# Autodesk Inventor assembly: Hotplate Assembly V01
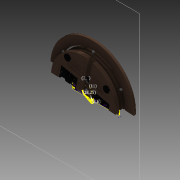
[picture p0: Inventor's stored thumbnail of the model, 180x180]
Saved by Autodesk Inventor 2015 (Build 190159000, 159)
## iProperties
Created: 2016-08-07
Part Number: Hotplate Assembly V01
Document SubType Name: Assembly
Designer: spichelh
Author: spichelh
## Documents named in this file (13)
- C:\Users\spichelh\Documents\GitHub\beta-hardware\Manufacturing Tools\PCB Reflow Hotplate V01\Hotplate Assembly V01.iam
- C:\Users\spichelh\Documents\GitHub\beta-hardware\Manufacturing Tools\PCB Reflow Hotplate V01\Ceramic Heating Element.ipt
- C:\Users\spichelh\Documents\GitHub\beta-hardware\Manufacturing Tools\PCB Reflow Hotplate V01\Hotplate Top 01.ipt
- C:\Users\spichelh\Documents\GitHub\beta-hardware\Manufacturing Tools\PCB Reflow Hotplate V01\HandleTop01.ipt
- C:\Users\spichelh\Documents\GitHub\beta-hardware\Manufacturing Tools\PCB Reflow Bracket V01\PCBBracket01.iam
- C:\Users\spichelh\Documents\GitHub\beta-hardware\Manufacturing Tools\PCB Reflow Hotplate V01\Hotplate Bottom 01.ipt
- C:\Users\spichelh\Documents\GitHub\beta-hardware\Manufacturing Tools\PCB Reflow Hotplate V01\Slippad.ipt
- C:\Users\spichelh\Documents\GitHub\beta-hardware\Manufacturing Tools\PCB Reflow Hotplate V01\HeatingElementHolder01.ipt
- C:\Users\spichelh\Documents\Inventor\Content Center Files\R2015\en-US\JIS B 1111(1)\JIS B 1111 - M2,5x5(1).ipt
- C:\Users\spichelh\Documents\Inventor\Content Center Files\R2015\en-US\ANSI B18.3.1M(1)\ANSI B18.3.1M - M2,5x0,45 x 4(2).ipt
- C:\Users\spichelh\Documents\GitHub\beta-hardware\Manufacturing Tools\PCB Reflow Hotplate V01\Imported Components\KFL08\KFL08.iam
- C:\Users\spichelh\Documents\GitHub\beta-hardware\Manufacturing Tools\PCB Reflow Hotplate V01\Cooler40x40.ipt
- C:\Users\spichelh\Documents\Inventor\Content Center Files\R2015\en-US\ANSI B18.3.1M(1)\ANSI B18.3.1M - M4x0,7 x 6(2).ipt
## Components (30 placed, 12 different names)
1. Ceramic Heating Element:1 — Mate:5, Mate:6, Mate:7
2. Hotplate Top 01:1 — Flush:1, Flush:2, Mate:1, Mate:2, Mate:3, Mate:4, Mate:5, Mate:6, Mate:7, Mate:8, Mate:9, Mate:10, Mate:11, Mate:12, Mate:13, Mate:14, Mate:15, Mate:16, Mate:18, Mate:19, Mate:21, Mate:32, Mate:33, Mate:34
3. Ceramic Heating Element:2 — Mate:8, Mate:9, Mate:10
4. Ceramic Heating Element:3 — Mate:11, Mate:12, Mate:13
5. Ceramic Heating Element:5 — Mate:14, Mate:15, Mate:16
6. Ceramic Heating Element:6 — Mate:1, Mate:2, Mate:3, Mate:20
7. HandleTop01:1 — Flush:1, Flush:2, Flush:3, Mate:32, Mate:36, Cylindrical:1
8. PCBBracket01:1 [sub-assembly] — Mate:4
9. Hotplate Bottom 01:1 — Mate:18, Mate:33, Mate:34, Mate:37, Mate:38, Mate:39, Mate:40, Mate:41, Mate:42, Mate:43, Mate:44, Rigid:5, Rigid:6, Rigid:7, Rigid:8, Mate:45, Mate:46
10. Slippad:1 — Mate:17, Rigid:5
11. Slippad:2 — Rigid:6
12. Slippad:3 — Rigid:7
13. Slippad:4 — Rigid:8
14. HeatingElementHolder01:1 — Mate:19, Mate:20, Mate:21, Mate:22, Mate:23, Mate:24, Mate:25, Mate:26, Mate:27, Mate:28, Mate:29, Mate:30, Mate:31
15. JIS B 1111 M2,5x5:1 — Mate:22, Mate:23
16. JIS B 1111 M2,5x5:2 — Mate:24, Mate:25
17. JIS B 1111 M2,5x5:3 — Mate:26, Mate:27
18. JIS B 1111 M2,5x5:4 — Mate:28, Mate:29
19. JIS B 1111 M2,5x5:5 — Mate:30, Mate:31
20. KFL08:1 [sub-assembly] — Mate:37, Mate:38, Mate:45, Mate:46, Mate:47, Mate:48, Mate:49, Mate:50
21. Cooler40x40:1 — Mate:42, Mate:43, Mate:44
22. Cooler40x40:2 — Mate:39, Mate:40, Mate:41
23. Broached Socket Head Cap Screw - Metric M4x0,7 x 6:1 — Mate:47, Mate:48
24. Broached Socket Head Cap Screw - Metric M4x0,7 x 6:2 — Mate:49, Mate:50
25. Broached Socket Head Cap Screw - Metric M2,5x0,45 x 4:2 — Mate:36, Cylindrical:1
26. Broached Socket Head Cap Screw - Metric M2,5x0,45 x 4:3
27. Broached Socket Head Cap Screw - Metric M2,5x0,45 x 4:4
28. Broached Socket Head Cap Screw - Metric M2,5x0,45 x 4:5
29. Broached Socket Head Cap Screw - Metric M2,5x0,45 x 4:6
30. Broached Socket Head Cap Screw - Metric M2,5x0,45 x 4:7
## Component patterns: (6 elements, first: Broached Socket Head Cap Screw - Metric M2,5x0,45 x 4:2)
## Relationships (57: Mate 49, WeldJoint 4, Flush 3, CylindricalJoint 1)
- Flush:1: Hotplate Top 01:1 ↔ HandleTop01:1
- Flush:2 (3 mm): Hotplate Top 01:1 ↔ HandleTop01:1
- Mate:1: Hotplate Top 01:1 ↔ Ceramic Heating Element:6
- Mate:2 (2 mm): Hotplate Top 01:1 ↔ Ceramic Heating Element:6
- Mate:3 (2 mm): Hotplate Top 01:1 ↔ Ceramic Heating Element:6
- Mate:4: Hotplate Top 01:1 ↔ PCBBracket01:1
- Mate:5: Ceramic Heating Element:1 ↔ Hotplate Top 01:1
- Mate:6 (2 mm): Ceramic Heating Element:1 ↔ Hotplate Top 01:1
- Mate:7 (2 mm): Ceramic Heating Element:1 ↔ Hotplate Top 01:1
- Mate:8: Hotplate Top 01:1 ↔ Ceramic Heating Element:2
- Mate:9 (2 mm): Hotplate Top 01:1 ↔ Ceramic Heating Element:2
- Mate:10 (2 mm): Hotplate Top 01:1 ↔ Ceramic Heating Element:2
- Mate:11: Hotplate Top 01:1 ↔ Ceramic Heating Element:3
- Mate:12 (2 mm): Hotplate Top 01:1 ↔ Ceramic Heating Element:3
- Mate:13 (2 mm): Hotplate Top 01:1 ↔ Ceramic Heating Element:3
- Mate:14: Hotplate Top 01:1 ↔ Ceramic Heating Element:5
- Mate:15 (2 mm): Hotplate Top 01:1 ↔ Ceramic Heating Element:5
- Mate:16 (2 mm): Hotplate Top 01:1 ↔ Ceramic Heating Element:5
- Mate:17: Slippad:1
- Mate:18: Hotplate Top 01:1 ↔ Hotplate Bottom 01:1
- Mate:19: Hotplate Top 01:1 ↔ HeatingElementHolder01:1
- Mate:20: Ceramic Heating Element:6 ↔ HeatingElementHolder01:1
- Mate:21: Hotplate Top 01:1 ↔ HeatingElementHolder01:1
- Mate:22: HeatingElementHolder01:1 ↔ JIS B 1111 M2,5x5:1
- Mate:23: HeatingElementHolder01:1 ↔ JIS B 1111 M2,5x5:1
- Mate:24: HeatingElementHolder01:1 ↔ JIS B 1111 M2,5x5:2
- Mate:25: HeatingElementHolder01:1 ↔ JIS B 1111 M2,5x5:2
- Mate:26: HeatingElementHolder01:1 ↔ JIS B 1111 M2,5x5:3
- Mate:27: HeatingElementHolder01:1 ↔ JIS B 1111 M2,5x5:3
- Mate:28: HeatingElementHolder01:1 ↔ JIS B 1111 M2,5x5:4
- Mate:29: HeatingElementHolder01:1 ↔ JIS B 1111 M2,5x5:4
- Mate:30: HeatingElementHolder01:1 ↔ JIS B 1111 M2,5x5:5
- Mate:31: HeatingElementHolder01:1 ↔ JIS B 1111 M2,5x5:5
- Flush:3: HandleTop01:1
- Mate:32: Hotplate Top 01:1 ↔ HandleTop01:1
- Mate:33: Hotplate Top 01:1 ↔ Hotplate Bottom 01:1
- Mate:34: Hotplate Top 01:1 ↔ Hotplate Bottom 01:1
- Mate:36: HandleTop01:1 ↔ Broached Socket Head Cap Screw - Metric M2,5x0,45 x 4:2
- Cylindrical:1: HandleTop01:1 ↔ Broached Socket Head Cap Screw - Metric M2,5x0,45 x 4:2
- Mate:37: Hotplate Bottom 01:1 ↔ KFL08:1
- Mate:38: Hotplate Bottom 01:1 ↔ KFL08:1
- Mate:39: Hotplate Bottom 01:1 ↔ Cooler40x40:2
- Mate:40 (1 mm): Hotplate Bottom 01:1 ↔ Cooler40x40:2
- Mate:41 (1 mm): Hotplate Bottom 01:1 ↔ Cooler40x40:2
- Mate:42: Hotplate Bottom 01:1 ↔ Cooler40x40:1
- Mate:43 (1 mm): Hotplate Bottom 01:1 ↔ Cooler40x40:1
- Mate:44 (1 mm): Hotplate Bottom 01:1 ↔ Cooler40x40:1
- Rigid:5 [WeldJoint]: Hotplate Bottom 01:1 ↔ Slippad:1
- Rigid:6 [WeldJoint]: Hotplate Bottom 01:1 ↔ Slippad:2
- Rigid:7 [WeldJoint]: Hotplate Bottom 01:1 ↔ Slippad:3
- Rigid:8 [WeldJoint]: Hotplate Bottom 01:1 ↔ Slippad:4
- Mate:45: Hotplate Bottom 01:1 ↔ KFL08:1
- Mate:46: Hotplate Bottom 01:1 ↔ KFL08:1
- Mate:47: KFL08:1 ↔ Broached Socket Head Cap Screw - Metric M4x0,7 x 6:1
- Mate:48: KFL08:1 ↔ Broached Socket Head Cap Screw - Metric M4x0,7 x 6:1
- Mate:49: KFL08:1 ↔ Broached Socket Head Cap Screw - Metric M4x0,7 x 6:2
- Mate:50: KFL08:1 ↔ Broached Socket Head Cap Screw - Metric M4x0,7 x 6:2
